# Autodesk Inventor assembly: Assembly1
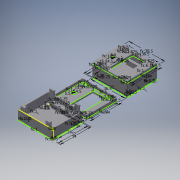
[picture p0: Inventor's stored thumbnail of the model, 180x180]
Saved by Autodesk Inventor 2019 (Build 230136000, 136)
## iProperties
Created: 2019-01-04
Part Number: Assembly1
Document SubType Name: Assembly
Designer: flato
Author: flato
## Documents named in this file (4)
- F:\Content creation\Projects\handheldWeatherStation\3D model\Inventor files\Assembly1.iam
- ViewModel.iam
- F:\Content creation\Projects\handheldWeatherStation\3D model\Inventor files\HandHeldWeatherStation housing.ipt
- F:\Content creation\Projects\handheldWeatherStation\3D model\Inventor files\Lid.ipt
## Components (4 placed, 2 different names)
1. HandHeldWeatherStation housing:1 — Mate:1, Mate:5, Mate:6
2. Lid:1 — Mate:2, Mate:3
3. HandHeldWeatherStation housing:2 — Mate:4
4. Lid:2 — Mate:5, Mate:6
## Relationships (6: Mate 6)
- Mate:1: HandHeldWeatherStation housing:1
- Mate:2: Lid:1
- Mate:3: Lid:1
- Mate:4: HandHeldWeatherStation housing:2
- Mate:5: HandHeldWeatherStation housing:1 ↔ Lid:2
- Mate:6: HandHeldWeatherStation housing:1 ↔ Lid:2
